# Autodesk Inventor assembly: Cage_connector_single_v06
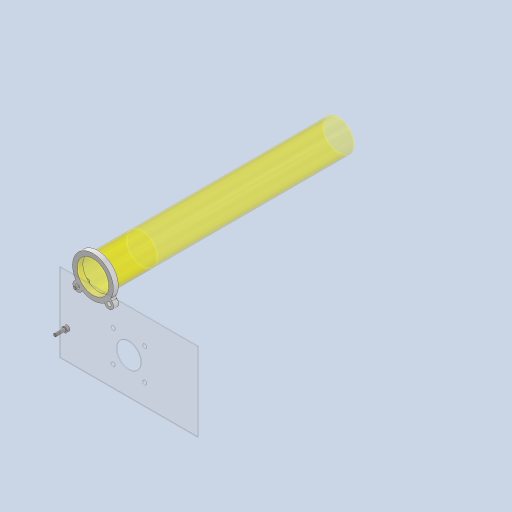
[picture p0: Inventor's stored thumbnail of the model, 512x512]
Saved by Autodesk Inventor 2024.4 (Build 284460030, 460C)
## iProperties
Created: 2026-03-25
Part Number: Cage_connector_single_v06
Document SubType Name: Assembly
Designer: tooles01
Author: tooles01
## iProperties of the stored document MemberDocs/xKrswxfkuLchbobh4Sdohgw0c4c
Created: 2026-03-25
Part Number: Cage_connector_single_v06
Document SubType Name: Assembly
Designer: tooles01
Author: tooles01
## iProperties of the stored document MemberDocs/xCn5q2qdhM0kstg35Nfetbfz4Yb
Created: 2026-03-25
Part Number: Cage_connector_single_v06
Document SubType Name: Assembly
Designer: tooles01
Author: tooles01
## iProperties of the stored document MemberDocs/xTpshylplA04gt0a0Slo1fy0eGb
Created: 2026-03-25
Part Number: Cage_connector_single_v06
Document SubType Name: Assembly
Designer: tooles01
Author: tooles01
## iProperties of the stored document MemberDocs/xPbgsdkdlFsqp1bfsCgcvfiahUc
Created: 2026-03-25
Part Number: Cage_connector_single_v06
Document SubType Name: Assembly
Designer: tooles01
Author: tooles01
## iProperties of the stored document MemberDocs/xY1fgm01cCsedmqhm1wevu01cQd
Created: 2026-03-25
Part Number: Cage_connector_single_v06
Document SubType Name: Assembly
Designer: tooles01
Author: tooles01
## Documents named in this file (12)
- C:\Users\tooles01\NYU Langone Health Dropbox\Shannon Toole\Shannon_Dropbox\Mar lab\RFID\CAD\Cage_connector\Cage_connector_single_v06.iam
- C:\Users\tooles01\NYU Langone Health Dropbox\Shannon Toole\Shannon_Dropbox\Mar lab\Inventor_Lib\M3 heat-set insert.ipt
- C:\Users\tooles01\Documents\Inventor\Content Center Files\R2024\en-US\AS 1420\AS 1420 - 1973 - M3 x 10.ipt
- C:\Users\tooles01\NYU Langone Health Dropbox\Shannon Toole\Shannon_Dropbox\Mar lab\Inventor_Lib\tube_5cm.ipt
- C:\Users\tooles01\NYU Langone Health Dropbox\Shannon Toole\Shannon_Dropbox\Mar lab\Inventor_Lib\tube_25cm.ipt
- C:\Users\tooles01\NYU Langone Health Dropbox\Shannon Toole\Shannon_Dropbox\Mar lab\Inventor_Lib\cage_wall_back.ipt
- C:\Users\tooles01\NYU Langone Health Dropbox\Shannon Toole\Shannon_Dropbox\Mar lab\RFID\CAD\Cage_connector\cage_inside_07.ipt
- C:\Users\tooles01\NYU Langone Health Dropbox\Shannon Toole\Shannon_Dropbox\Mar lab\RFID\CAD\lib\M3 heat-set insert.ipt
- C:\Users\tooles01\NYU Langone Health Dropbox\Shannon Toole\Shannon_Dropbox\Mar lab\RFID\CAD\lib\tube_5cm.ipt
- C:\Users\tooles01\NYU Langone Health Dropbox\Shannon Toole\Shannon_Dropbox\Mar lab\RFID\CAD\lib\tube_25cm.ipt
- C:\Users\tooles01\NYU Langone Health Dropbox\Shannon Toole\Shannon_Dropbox\Mar lab\RFID\CAD\lib\cage_wall_holes.ipt
- C:\Users\tooles01\NYU Langone Health Dropbox\Shannon Toole\Shannon_Dropbox\Mar lab\RFID\CAD\Cage_connector\cage_inside_05.ipt
## Components (8 placed, 6 different names)
1. cage_wall_back:1 — cage_inside to wall:1, screw to wall:1, screw to wall:2
2. cage_inside_07:1 — cage_inside to wall:1, heat-set to cage_inside:1, heat-set to cage_inside:2, short tube to cage_inside:1, long tube to cage_inside:1
3. tube_5cm:1 — short tube to cage_inside:1
4. tube_25cm:1 — long tube to cage_inside:1
5. M3 heat-set insert:1 — heat-set to cage_inside:1, screw to heat-set:1
6. M3 heat-set insert:2 — heat-set to cage_inside:2, screw to heat-set:2
7. AS 1420 - Metric M3 x 10:1 — screw to heat-set:1, screw to wall:1
8. AS 1420 - Metric M3 x 10:2 — screw to heat-set:2, screw to wall:2
## Relationships (9: Insert 7, Mate 2)
- cage_inside to wall:1 [Insert]: cage_wall_back:1 ↔ cage_inside_07:1
- short tube to cage_inside:1 [Insert]: cage_inside_07:1 ↔ tube_5cm:1
- long tube to cage_inside:1 [Insert]: cage_inside_07:1 ↔ tube_25cm:1
- heat-set to cage_inside:1 [Insert]: cage_inside_07:1 ↔ M3 heat-set insert:1
- heat-set to cage_inside:2 [Insert]: cage_inside_07:1 ↔ M3 heat-set insert:2
- screw to heat-set:1 [Mate]: M3 heat-set insert:1 ↔ AS 1420 - Metric M3 x 10:1
- screw to heat-set:2 [Mate]: M3 heat-set insert:2 ↔ AS 1420 - Metric M3 x 10:2
- screw to wall:1 [Insert]: cage_wall_back:1 ↔ AS 1420 - Metric M3 x 10:1
- screw to wall:2 [Insert]: cage_wall_back:1 ↔ AS 1420 - Metric M3 x 10:2
